# Autodesk Inventor assembly: SXRL24-150 v1
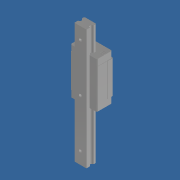
[picture p0: Inventor's stored thumbnail of the model, 180x180]
Saved by Autodesk Inventor 2020 (Build 240168000, 168)
## iProperties
Created: 2021-08-17
Part Number: SXRL24-150 v1
Document SubType Name: Assembly
Designer: ken113
Author: ken113
## Documents named in this file (3)
- D:\Document\Github\Vibration_Generator\Parts\Sample\SXRL24-150 v1.iam
- D:\Document\Github\Vibration_Generator\Parts\Sample\_SXRL24-150_r.ipt
- D:\Document\Github\Vibration_Generator\Parts\Sample\_SXRL24-150_b.ipt
## Components (2 placed, 2 different names)
1. _SXRL24-150_r:1 — メイト:1, メイト:2
2. _SXRL24-150_b:1 — メイト:1, メイト:2
## Relationships (2: Mate 2)
- メイト:1 [Mate]: _SXRL24-150_r:1 ↔ _SXRL24-150_b:1
- メイト:2 [Mate]: _SXRL24-150_r:1 ↔ _SXRL24-150_b:1
